# Autodesk Inventor assembly: Camera_assembly 2
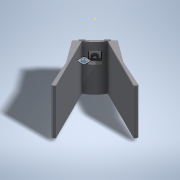
[picture p0: Inventor's stored thumbnail of the model, 180x180]
Saved by Autodesk Inventor 2022 (Build 260153000, 153)
## iProperties
Created: 2023-04-06
Part Number: Camera_assembly 2
Document SubType Name: Assembly
Designer: zarek
Author: zarek
## Documents named in this file (3)
- C:\Users\zarek\OneDrive\Desktop\Random New Stuff\SPB\Camera_assembly 2.iam
- C:\Users\zarek\OneDrive\Desktop\Random New Stuff\SPB\Camera_Holder - LED.ipt
- C:\Users\zarek\OneDrive\Desktop\Random New Stuff\SPB\Camera & Angle.iam
## Components (2 placed, 2 different names)
1. Camera_Holder - LED:1 — Rotational:1
2. Camera & Angle:1 [sub-assembly] — Rotational:1
## Relationships (1: RevoluteJoint 1)
- Rotational:1 [RevoluteJoint] (-5 mm): Camera_Holder - LED:1 ↔ Camera & Angle:1
